# Autodesk Inventor assembly: LCDassembly
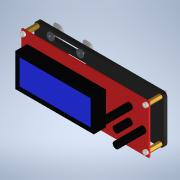
[picture p0: Inventor's stored thumbnail of the model, 180x180]
Saved by Autodesk Inventor 2020.2 (Build 242310000, 310)
## iProperties
Created: 2020-08-24
Part Number: LCDassembly
Document SubType Name: Assembly
Designer: JK
Author: JK
## Documents named in this file (7)
- C:\Users\JK\Documents\Inventor\Anet Upgrade\LCDassembly.iam
- C:\Users\JK\Documents\Inventor\Anet Upgrade\LCDmount.ipt
- C:\Users\JK\Documents\Inventor\Anet Upgrade\LCDScreen.ipt
- C:\Users\JK\Documents\Inventor\Anet Upgrade\M5x12BoltFlatHead.ipt
- C:\Users\JK\Documents\Inventor\Anet Upgrade\T_Slot_Nut_Dropin_3030m5ipt.ipt
- C:\Users\JK\Documents\Inventor\Anet Upgrade\HexagonalSpacer.ipt
- C:\Users\JK\Documents\Inventor\Anet Upgrade\M3x10.ipt
## Components (18 placed, 6 different names)
1. LCDmount:1 — Mate:1, Mate:2, Mate:5, Mate:6, Mate:7, Mate:8, Mate:9, Mate:10, Mate:11, Mate:12, Mate:13, Angle:1, Mate:19, Mate:20, Mate:21, Mate:22, Mate:24
2. LCDScreen:1 — Mate:1, Mate:2, Mate:14, Mate:15, Mate:16, Mate:17, Mate:18, Mate:23
3. M5x12BoltFlatHead:1 — Flush:1, Mate:4
4. M5x12BoltFlatHead:2 — Flush:1, Mate:3
5. T_Slot_Nut_Dropin_3030m5ipt:1 — Mate:3, Flush:2, Mate:8, Flush:3
6. T_Slot_Nut_Dropin_3030m5ipt:2 — Mate:4, Flush:2, Mate:5, Mate:6, Mate:7, Flush:3
7. HexagonalSpacer:1 — Mate:10, Flush:4, Flush:8
8. HexagonalSpacer:2 — Mate:9, Mate:13, Flush:4, Flush:5, Flush:7
9. HexagonalSpacer:3 — Mate:11, Flush:5, Flush:6, Mate:14, Flush:7
10. HexagonalSpacer:4 — Mate:12, Flush:6, Flush:8, Angle:1
11. M3x10:1 — Mate:21, Flush:14
12. M3x10:2 — Mate:20, Flush:12, Flush:13
13. M3x10:3 — Mate:18, Flush:9
14. M3x10:4 — Mate:17, Flush:11
15. M3x10:5 — Mate:19, Mate:24, Flush:12
16. M3x10:6 — Mate:15, Mate:23, Flush:9, Flush:10
17. M3x10:7 — Mate:16, Flush:10, Flush:11
18. M3x10:8 — Mate:22, Flush:13, Flush:14
## Relationships (39: Mate 24, Flush 14, Angle 1)
- Mate:1: LCDmount:1 ↔ LCDScreen:1
- Mate:2: LCDmount:1 ↔ LCDScreen:1
- Flush:1: M5x12BoltFlatHead:1 ↔ M5x12BoltFlatHead:2
- Mate:3: M5x12BoltFlatHead:2 ↔ T_Slot_Nut_Dropin_3030m5ipt:1
- Mate:4: M5x12BoltFlatHead:1 ↔ T_Slot_Nut_Dropin_3030m5ipt:2
- Flush:2: T_Slot_Nut_Dropin_3030m5ipt:1 ↔ T_Slot_Nut_Dropin_3030m5ipt:2
- Mate:5 (-1.5 mm): LCDmount:1 ↔ T_Slot_Nut_Dropin_3030m5ipt:2
- Mate:6: LCDmount:1 ↔ T_Slot_Nut_Dropin_3030m5ipt:2
- Mate:7: LCDmount:1 ↔ T_Slot_Nut_Dropin_3030m5ipt:2
- Mate:8: LCDmount:1 ↔ T_Slot_Nut_Dropin_3030m5ipt:1
- Flush:3: T_Slot_Nut_Dropin_3030m5ipt:1 ↔ T_Slot_Nut_Dropin_3030m5ipt:2
- Mate:9: LCDmount:1 ↔ HexagonalSpacer:2
- Mate:10: LCDmount:1 ↔ HexagonalSpacer:1
- Mate:11: LCDmount:1 ↔ HexagonalSpacer:3
- Mate:12: LCDmount:1 ↔ HexagonalSpacer:4
- Mate:13: LCDmount:1 ↔ HexagonalSpacer:2
- Flush:4: HexagonalSpacer:1 ↔ HexagonalSpacer:2
- Flush:5: HexagonalSpacer:2 ↔ HexagonalSpacer:3
- Flush:6: HexagonalSpacer:3 ↔ HexagonalSpacer:4
- Mate:14: LCDScreen:1 ↔ HexagonalSpacer:3
- Flush:7: HexagonalSpacer:2 ↔ HexagonalSpacer:3
- Flush:8: HexagonalSpacer:1 ↔ HexagonalSpacer:4
- Angle:1 (0 deg): LCDmount:1 ↔ HexagonalSpacer:4
- Mate:15: LCDScreen:1 ↔ M3x10:6
- Mate:16: LCDScreen:1 ↔ M3x10:7
- Mate:17: LCDScreen:1 ↔ M3x10:4
- Mate:18: LCDScreen:1 ↔ M3x10:3
- Mate:19: LCDmount:1 ↔ M3x10:5
- Mate:20: LCDmount:1 ↔ M3x10:2
- Mate:21: LCDmount:1 ↔ M3x10:1
- Mate:22: LCDmount:1 ↔ M3x10:8
- Mate:23: LCDScreen:1 ↔ M3x10:6
- Flush:9: M3x10:3 ↔ M3x10:6
- Flush:10: M3x10:6 ↔ M3x10:7
- Flush:11: M3x10:4 ↔ M3x10:7
- Mate:24: LCDmount:1 ↔ M3x10:5
- Flush:12: M3x10:2 ↔ M3x10:5
- Flush:13: M3x10:2 ↔ M3x10:8
- Flush:14: M3x10:1 ↔ M3x10:8
